# Autodesk Inventor assembly: PCB1_23.12
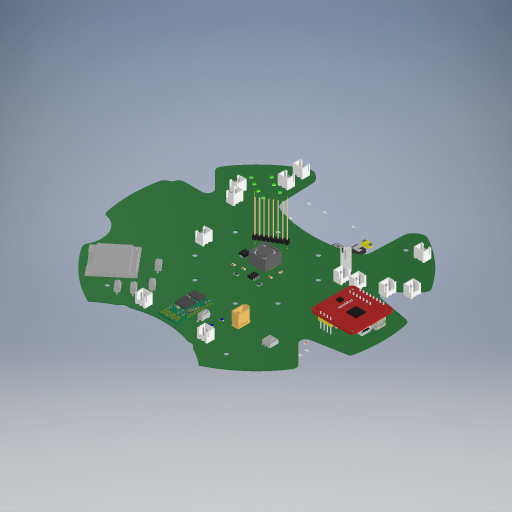
[picture p0: Inventor's stored thumbnail of the model, 512x512]
Saved by Autodesk Inventor 2023 (Build 270158000, 158)
## iProperties
Company: Open CASCADE
Created: 2024-12-23
Part Number: PCB1_23.12
Description: Open CASCADE Model
Document SubType Name: Assembly
Designer: Ivan
Authority: Unknown
Mass: 19.3363 g
Surface Area: 696.783 cm^2
Volume: 19.8929 cm^3
Density: 0.972022 g/cm^3
Sending System: Open CASCADE 7.5
Preprocessor: Open CASCADE STEP processor 7.5
Title: Open CASCADE Shape Model
Author: Author
## Documents named in this file (133)
- C:\!projects\DASH-\3D\Dash-V1\motherboard\PCB2\PCB1_23.12.iam
- C:\!projects\DASH-\3D\Dash-V1\motherboard\PCB2\Board.iam
- C:\!projects\DASH-\3D\Dash-V1\motherboard\PCB2\D1_1.iam
- C:\!projects\DASH-\3D\Dash-V1\motherboard\PCB2\+5V.iam
- C:\!projects\DASH-\3D\Dash-V1\motherboard\PCB2\+3V3.iam
- C:\!projects\DASH-\3D\Dash-V1\motherboard\PCB2\C20.iam
- C:\!projects\DASH-\3D\Dash-V1\motherboard\PCB2\C19.iam
- C:\!projects\DASH-\3D\Dash-V1\motherboard\PCB2\C18.iam
- C:\!projects\DASH-\3D\Dash-V1\motherboard\PCB2\C13.iam
- C:\!projects\DASH-\3D\Dash-V1\motherboard\PCB2\C3_4.iam
- C:\!projects\DASH-\3D\Dash-V1\motherboard\PCB2\C3_3.iam
- C:\!projects\DASH-\3D\Dash-V1\motherboard\PCB2\C3_2.iam
- C:\!projects\DASH-\3D\Dash-V1\motherboard\PCB2\C3_1.iam
- C:\!projects\DASH-\3D\Dash-V1\motherboard\PCB2\C2_4.iam
- C:\!projects\DASH-\3D\Dash-V1\motherboard\PCB2\C2_3.iam
- C:\!projects\DASH-\3D\Dash-V1\motherboard\PCB2\C2_2.iam
- C:\!projects\DASH-\3D\Dash-V1\motherboard\PCB2\C2_1.iam
- C:\!projects\DASH-\3D\Dash-V1\motherboard\PCB2\C12.iam
- C:\!projects\DASH-\3D\Dash-V1\motherboard\PCB2\sen1_power.iam
- C:\!projects\DASH-\3D\Dash-V1\motherboard\PCB2\sen2_power.iam
- C:\!projects\DASH-\3D\Dash-V1\motherboard\PCB2\sen2.iam
- C:\!projects\DASH-\3D\Dash-V1\motherboard\PCB2\dribler_data.iam
- C:\!projects\DASH-\3D\Dash-V1\motherboard\PCB2\dribler_power.iam
- C:\!projects\DASH-\3D\Dash-V1\motherboard\PCB2\C9.iam
- C:\!projects\DASH-\3D\Dash-V1\motherboard\PCB2\C10.iam
- C:\!projects\DASH-\3D\Dash-V1\motherboard\PCB2\C11.iam
- C:\!projects\DASH-\3D\Dash-V1\motherboard\PCB2\C14.iam
- C:\!projects\DASH-\3D\Dash-V1\motherboard\PCB2\C15.iam
- C:\!projects\DASH-\3D\Dash-V1\motherboard\PCB2\C16.iam
- C:\!projects\DASH-\3D\Dash-V1\motherboard\PCB2\C17.iam
- C:\!projects\DASH-\3D\Dash-V1\motherboard\PCB2\C5.iam
- C:\!projects\DASH-\3D\Dash-V1\motherboard\PCB2\C6.iam
- C:\!projects\DASH-\3D\Dash-V1\motherboard\PCB2\C7.iam
- C:\!projects\DASH-\3D\Dash-V1\motherboard\PCB2\C8.iam
- C:\!projects\DASH-\3D\Dash-V1\motherboard\PCB2\DA1.iam
- C:\!projects\DASH-\3D\Dash-V1\motherboard\PCB2\L1.iam
- C:\!projects\DASH-\3D\Dash-V1\motherboard\PCB2\R32.iam
- C:\!projects\DASH-\3D\Dash-V1\motherboard\PCB2\R33.iam
- C:\!projects\DASH-\3D\Dash-V1\motherboard\PCB2\R34.iam
- C:\!projects\DASH-\3D\Dash-V1\motherboard\PCB2\R35.iam
- C:\!projects\DASH-\3D\Dash-V1\motherboard\PCB2\R36.iam
- C:\!projects\DASH-\3D\Dash-V1\motherboard\PCB2\R37.iam
- C:\!projects\DASH-\3D\Dash-V1\motherboard\PCB2\R38.iam
- C:\!projects\DASH-\3D\Dash-V1\motherboard\PCB2\R39.iam
- C:\!projects\DASH-\3D\Dash-V1\motherboard\PCB2\R40.iam
- C:\!projects\DASH-\3D\Dash-V1\motherboard\PCB2\R17.iam
- C:\!projects\DASH-\3D\Dash-V1\motherboard\PCB2\R18.iam
- C:\!projects\DASH-\3D\Dash-V1\motherboard\PCB2\R19.iam
- C:\!projects\DASH-\3D\Dash-V1\motherboard\PCB2\R20.iam
- C:\!projects\DASH-\3D\Dash-V1\motherboard\PCB2\R21.iam
- C:\!projects\DASH-\3D\Dash-V1\motherboard\PCB2\R22.iam
- C:\!projects\DASH-\3D\Dash-V1\motherboard\PCB2\R23.iam
- C:\!projects\DASH-\3D\Dash-V1\motherboard\PCB2\R24.iam
- C:\!projects\DASH-\3D\Dash-V1\motherboard\PCB2\R25.iam
- C:\!projects\DASH-\3D\Dash-V1\motherboard\PCB2\R26.iam
- C:\!projects\DASH-\3D\Dash-V1\motherboard\PCB2\R27.iam
- C:\!projects\DASH-\3D\Dash-V1\motherboard\PCB2\R28.iam
- C:\!projects\DASH-\3D\Dash-V1\motherboard\PCB2\R29.iam
- C:\!projects\DASH-\3D\Dash-V1\motherboard\PCB2\R30.iam
- C:\!projects\DASH-\3D\Dash-V1\motherboard\PCB2\R31.iam
- C:\!projects\DASH-\3D\Dash-V1\motherboard\PCB2\Power.iam
- C:\!projects\DASH-\3D\Dash-V1\motherboard\PCB2\Down.iam
- C:\!projects\DASH-\3D\Dash-V1\motherboard\PCB2\Reset.iam
- C:\!projects\DASH-\3D\Dash-V1\motherboard\PCB2\Enter.iam
- C:\!projects\DASH-\3D\Dash-V1\motherboard\PCB2\Up.iam
- C:\!projects\DASH-\3D\Dash-V1\motherboard\PCB2\U2.iam
- C:\!projects\DASH-\3D\Dash-V1\motherboard\PCB2\VD12.iam
- C:\!projects\DASH-\3D\Dash-V1\motherboard\PCB2\+12V.iam
- C:\!projects\DASH-\3D\Dash-V1\motherboard\PCB2\Led1.iam
- C:\!projects\DASH-\3D\Dash-V1\motherboard\PCB2\Led2.iam
- C:\!projects\DASH-\3D\Dash-V1\motherboard\PCB2\Led3.iam
- C:\!projects\DASH-\3D\Dash-V1\motherboard\PCB2\Led4.iam
- C:\!projects\DASH-\3D\Dash-V1\motherboard\PCB2\VD13.iam
- C:\!projects\DASH-\3D\Dash-V1\motherboard\PCB2\VT3.iam
- C:\!projects\DASH-\3D\Dash-V1\motherboard\PCB2\VT4.iam
- C:\!projects\DASH-\3D\Dash-V1\motherboard\PCB2\VT5.iam
- C:\!projects\DASH-\3D\Dash-V1\motherboard\PCB2\X1.iam
- C:\!projects\DASH-\3D\Dash-V1\motherboard\PCB2\D2_2.iam
- C:\!projects\DASH-\3D\Dash-V1\motherboard\PCB2\D2_3.iam
- C:\!projects\DASH-\3D\Dash-V1\motherboard\PCB2\D1_3.iam
- C:\!projects\DASH-\3D\Dash-V1\motherboard\PCB2\D2_1.iam
- C:\!projects\DASH-\3D\Dash-V1\motherboard\PCB2\D1_2.iam
- C:\!projects\DASH-\3D\Dash-V1\motherboard\PCB2\R9_1.iam
- C:\!projects\DASH-\3D\Dash-V1\motherboard\PCB2\R9_2.iam
- C:\!projects\DASH-\3D\Dash-V1\motherboard\PCB2\R9_3.iam
- C:\!projects\DASH-\3D\Dash-V1\motherboard\PCB2\R9_4.iam
- C:\!projects\DASH-\3D\Dash-V1\motherboard\PCB2\R8_1.iam
- C:\!projects\DASH-\3D\Dash-V1\motherboard\PCB2\R8_2.iam
- C:\!projects\DASH-\3D\Dash-V1\motherboard\PCB2\R8_3.iam
- C:\!projects\DASH-\3D\Dash-V1\motherboard\PCB2\R7_1.iam
- C:\!projects\DASH-\3D\Dash-V1\motherboard\PCB2\R7_2.iam
- C:\!projects\DASH-\3D\Dash-V1\motherboard\PCB2\R7_3.iam
- C:\!projects\DASH-\3D\Dash-V1\motherboard\PCB2\R6_1.iam
- C:\!projects\DASH-\3D\Dash-V1\motherboard\PCB2\R6_2.iam
- C:\!projects\DASH-\3D\Dash-V1\motherboard\PCB2\R6_3.iam
- C:\!projects\DASH-\3D\Dash-V1\motherboard\PCB2\Motor4.iam
- C:\!projects\DASH-\3D\Dash-V1\motherboard\PCB2\Motor3.iam
- C:\!projects\DASH-\3D\Dash-V1\motherboard\PCB2\Motor2.iam
- C:\!projects\DASH-\3D\Dash-V1\motherboard\PCB2\Motor1.iam
- C:\!projects\DASH-\3D\Dash-V1\motherboard\PCB2\VT2.iam
- C:\!projects\DASH-\3D\Dash-V1\motherboard\PCB2\VT1.iam
- C:\!projects\DASH-\3D\Dash-V1\motherboard\PCB2\VD3.iam
- C:\!projects\DASH-\3D\Dash-V1\motherboard\PCB2\R16.iam
- C:\!projects\DASH-\3D\Dash-V1\motherboard\PCB2\R15.iam
- C:\!projects\DASH-\3D\Dash-V1\motherboard\PCB2\R14.iam
- C:\!projects\DASH-\3D\Dash-V1\motherboard\PCB2\R13.iam
- C:\!projects\DASH-\3D\Dash-V1\motherboard\PCB2\R12.iam
- C:\!projects\DASH-\3D\Dash-V1\motherboard\PCB2\R11.iam
- C:\!projects\DASH-\3D\Dash-V1\motherboard\PCB2\C4.iam
- C:\!projects\DASH-\3D\Dash-V1\motherboard\PCB2\Sol2.iam
- C:\!projects\DASH-\3D\Dash-V1\motherboard\PCB2\Sol1.iam
- C:\!projects\DASH-\3D\Dash-V1\motherboard\PCB2\Cap.iam
- C:\!projects\DASH-\3D\Dash-V1\motherboard\PCB2\IRS4427.iam
- C:\!projects\DASH-\3D\Dash-V1\motherboard\PCB2\VD2.iam
- C:\!projects\DASH-\3D\Dash-V1\motherboard\PCB2\VD1.iam
- C:\!projects\DASH-\3D\Dash-V1\motherboard\PCB2\R5.iam
- C:\!projects\DASH-\3D\Dash-V1\motherboard\PCB2\R4.iam
- C:\!projects\DASH-\3D\Dash-V1\motherboard\PCB2\R3.iam
- C:\!projects\DASH-\3D\Dash-V1\motherboard\PCB2\R2.iam
- C:\!projects\DASH-\3D\Dash-V1\motherboard\PCB2\R1.iam
- C:\!projects\DASH-\3D\Dash-V1\motherboard\PCB2\open_MV.iam
- C:\!projects\DASH-\3D\Dash-V1\motherboard\PCB2\R8_4.iam
- C:\!projects\DASH-\3D\Dash-V1\motherboard\PCB2\R7_4.iam
- C:\!projects\DASH-\3D\Dash-V1\motherboard\PCB2\R6_4.iam
- C:\!projects\DASH-\3D\Dash-V1\motherboard\PCB2\D2_4.iam
- C:\!projects\DASH-\3D\Dash-V1\motherboard\PCB2\D1_4.iam
- C:\!projects\DASH-\3D\Dash-V1\motherboard\PCB2\VD4.iam
- C:\!projects\DASH-\3D\Dash-V1\motherboard\PCB2\SB1.iam
- C:\!projects\DASH-\3D\Dash-V1\motherboard\PCB2\OLED_SPI1.iam
- C:\!projects\DASH-\3D\Dash-V1\motherboard\PCB2\IC1.iam
- C:\!projects\DASH-\3D\Dash-V1\motherboard\PCB2\HC1.iam
- C:\!projects\DASH-\3D\Dash-V1\motherboard\PCB2\C1.iam
- C:\!projects\DASH-\3D\Dash-V1\step\lpls\DS1021_black_1x04p_100mil_Type43_rev1.0.ipt
## Components (133 placed, 132 different names)
1. Board_2 [sub-assembly] — Совмещение:11, Совмещение:20, Совмещение:22, Совмещение:23, Совмещение:24, Совмещение:25
2. D1_1_15 [sub-assembly]
3. +5V_17 [sub-assembly]
4. +3V3_19 [sub-assembly]
5. C20_21 [sub-assembly]
6. C19_23 [sub-assembly]
7. C18_25 [sub-assembly]
8. C13_27 [sub-assembly]
9. C3_4_29 [sub-assembly]
10. C3_3_31 [sub-assembly]
11. C3_2_33 [sub-assembly]
12. C3_1_35 [sub-assembly]
13. C2_4_37 [sub-assembly]
14. C2_3_39 [sub-assembly]
15. C2_2_41 [sub-assembly]
16. C2_1_43 [sub-assembly]
17. C12_45 [sub-assembly]
18. sen1_power_47 [sub-assembly] — Заподлицо:3
19. sen2_power_49 [sub-assembly]
20. sen2_53 [sub-assembly]
21. dribler_data_55 [sub-assembly] — Совмещение:25
22. dribler_power_57 [sub-assembly] — Заподлицо:3
23. C9_59 [sub-assembly]
24. C10_61 [sub-assembly]
25. C11_63 [sub-assembly]
26. C14_65 [sub-assembly]
27. C15_67 [sub-assembly]
28. C16_69 [sub-assembly]
29. C17_71 [sub-assembly]
30. C5_73 [sub-assembly]
31. C6_75 [sub-assembly]
32. C7_77 [sub-assembly]
33. C8_79 [sub-assembly]
34. DA1_81 [sub-assembly]
35. L1_83 [sub-assembly]
36. R32_85 [sub-assembly]
37. R33_87 [sub-assembly]
38. R34_89 [sub-assembly]
39. R35_91 [sub-assembly]
40. R36_93 [sub-assembly]
41. R37_95 [sub-assembly]
42. R38_97 [sub-assembly]
43. R39_99 [sub-assembly]
44. R40_101 [sub-assembly]
45. R17_103 [sub-assembly]
46. R18_105 [sub-assembly]
47. R19_107 [sub-assembly]
48. R20_109 [sub-assembly]
49. R21_111 [sub-assembly]
50. R22_113 [sub-assembly]
51. R23_115 [sub-assembly]
52. R24_117 [sub-assembly]
53. R25_119 [sub-assembly]
54. R26_121 [sub-assembly]
55. R27_123 [sub-assembly]
56. R28_125 [sub-assembly]
57. R29_127 [sub-assembly]
58. R30_129 [sub-assembly]
59. R31_131 [sub-assembly]
60. Power_133 [sub-assembly]
61. Down_135 [sub-assembly]
62. Reset_137 [sub-assembly]
63. Enter_139 [sub-assembly]
64. Up_141 [sub-assembly]
65. U2_143 [sub-assembly]
66. VD12_145 [sub-assembly]
67. +12V_147 [sub-assembly]
68. Led1_149 [sub-assembly]
69. Led2_151 [sub-assembly]
70. Led3_153 [sub-assembly]
71. Led4_155 [sub-assembly]
72. VD13_157 [sub-assembly]
73. VT3_204 [sub-assembly]
74. VT4_206 [sub-assembly]
75. VT5_209 [sub-assembly]
76. X1_214 [sub-assembly]
77. D2_2_216 [sub-assembly]
78. D2_3_218 [sub-assembly]
79. D1_3_220 [sub-assembly]
80. D2_1_222 [sub-assembly]
81. D1_2_224 [sub-assembly]
82. R9_1_226 [sub-assembly]
83. R9_2_228 [sub-assembly]
84. R9_3_230 [sub-assembly]
85. R9_4_232 [sub-assembly]
86. R8_1_234 [sub-assembly]
87. R8_2_236 [sub-assembly]
88. R8_3_238 [sub-assembly]
89. R7_1_240 [sub-assembly]
90. R7_2_242 [sub-assembly]
91. R7_3_244 [sub-assembly]
92. R6_1_246 [sub-assembly]
93. R6_2_248 [sub-assembly]
94. R6_3_250 [sub-assembly]
95. Motor4_252 [sub-assembly]
96. Motor3_254 [sub-assembly]
97. Motor2_256 [sub-assembly]
98. Motor1_258 [sub-assembly]
99. VT2_267 [sub-assembly]
100. VT1_276 [sub-assembly]
101. VD3_278 [sub-assembly]
102. R16_280 [sub-assembly]
103. R15_282 [sub-assembly]
104. R14_284 [sub-assembly]
105. R13_286 [sub-assembly]
106. R12_288 [sub-assembly]
107. R11_290 [sub-assembly]
108. C4_292 [sub-assembly]
109. Sol2_294 [sub-assembly]
110. Sol1_296 [sub-assembly]
111. Cap_298 [sub-assembly]
112. IRS4427_300 [sub-assembly]
113. VD2_302 [sub-assembly]
114. VD1_304 [sub-assembly]
115. R5_306 [sub-assembly]
116. R4_308 [sub-assembly]
117. R3_310 [sub-assembly]
118. R2_312 [sub-assembly]
119. R1_314 [sub-assembly]
120. open_MV_316 [sub-assembly]
121. R8_4_320 [sub-assembly]
122. R7_4_322 [sub-assembly]
123. R6_4_324 [sub-assembly]
124. D2_4_326 [sub-assembly]
125. D1_4_328 [sub-assembly]
126. VD4_330 [sub-assembly]
127. SB1_332 [sub-assembly]
128. OLED_SPI1_334 [sub-assembly]
129. IC1_336 [sub-assembly]
130. HC1_338 [sub-assembly]
131. C1_340 [sub-assembly]
132. DS1021_black_1x04p_100mil_Type43_rev1.0:1 — Заподлицо:1, Заподлицо:2, Совмещение:21, Совмещение:23, Совмещение:24
133. DS1021_black_1x04p_100mil_Type43_rev1.0:2 — Заподлицо:1, Заподлицо:2, Совмещение:21, Совмещение:22
## Relationships (14: Mate 11, Flush 3)
- Совмещение:9 [Mate]
- Совмещение:10 [Mate]
- Совмещение:11 [Mate]: Board_2
- Совмещение:18 [Mate]
- Совмещение:19 [Mate]
- Совмещение:20 [Mate]: Board_2
- Заподлицо:1 [Flush]: DS1021_black_1x04p_100mil_Type43_rev1.0:1 ↔ DS1021_black_1x04p_100mil_Type43_rev1.0:2
- Заподлицо:2 [Flush]: DS1021_black_1x04p_100mil_Type43_rev1.0:1 ↔ DS1021_black_1x04p_100mil_Type43_rev1.0:2
- Совмещение:21 [Mate]: DS1021_black_1x04p_100mil_Type43_rev1.0:1 ↔ DS1021_black_1x04p_100mil_Type43_rev1.0:2
- Совмещение:22 [Mate]: Board_2 ↔ DS1021_black_1x04p_100mil_Type43_rev1.0:2
- Совмещение:23 [Mate]: Board_2 ↔ DS1021_black_1x04p_100mil_Type43_rev1.0:1
- Совмещение:24 [Mate]: Board_2 ↔ DS1021_black_1x04p_100mil_Type43_rev1.0:1
- Совмещение:25 [Mate]: Board_2 ↔ dribler_data_55
- Заподлицо:3 [Flush]: sen1_power_47 ↔ dribler_power_57
